# Autodesk Inventor assembly: All Assembly
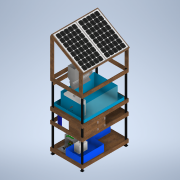
[picture p0: Inventor's stored thumbnail of the model, 180x180]
Saved by Autodesk Inventor 2020 (Build 240168000, 168)
## iProperties
Created: 2020-06-27
Part Number: All Assembly
Document SubType Name: Assembly
Designer: Abbas
Author: Abbas
## Documents named in this file (22)
- C:\Users\LENOVO\Desktop\Graduation Project\Fish Farming Unit\All Assembly\All Assembly.iam
- C:\Users\LENOVO\Desktop\Graduation Project\Fish Farming Unit\tub floor\tub floor 1.ipt
- C:\Users\LENOVO\Desktop\Graduation Project\Fish Farming Unit\tub floor\tub floor 2.ipt
- C:\Users\LENOVO\Desktop\Graduation Project\Fish Farming Unit\metal supporter\metal supporter.ipt
- C:\Users\LENOVO\Desktop\Graduation Project\Fish Farming Unit\Tub\tub_assembled.iam
- C:\Users\LENOVO\Desktop\Graduation Project\Fish Farming Unit\solar panels holder\solar panels holder 2.ipt
- C:\Users\LENOVO\Desktop\Graduation Project\Fish Farming Unit\Solar Panels With Holder\Solar Panels With Holder.iam
- C:\Users\LENOVO\Desktop\Graduation Project\Fish Farming Unit\foodstorage\Assembly1.iam
- C:\Users\LENOVO\Desktop\Graduation Project\Fish Farming Unit\tub floor\tub floor 3.ipt
- C:\Users\LENOVO\Desktop\Graduation Project\Fish Farming Unit\Water Loop Components\Ammonia Filter.iam
- C:\Users\LENOVO\Desktop\Graduation Project\Fish Farming Unit\Middle Floor\Middle Floor.ipt
- C:\Users\LENOVO\Desktop\Graduation Project\Fish Farming Unit\Sensors\NTC Thermistor\NTC thermistor.iam
- C:\Users\LENOVO\Desktop\Graduation Project\Fish Farming Unit\Sensors\ph-sensor-1.snapshot.1\PH_Probe.iam
- C:\Users\LENOVO\Desktop\Graduation Project\Fish Farming Unit\Water Loop Components\ammonia filter bracket.ipt
- C:\Users\LENOVO\Desktop\Graduation Project\Fish Farming Unit\feeding tank bracket\feeding tank bracket.ipt
- C:\Users\LENOVO\Desktop\Graduation Project\Fish Farming Unit\Tub Sensors Holder\Sensors Holder V3.ipt
- C:\Users\LENOVO\Desktop\Graduation Project\Fish Farming Unit\Pump System\Pump System.iam
- C:\Users\LENOVO\Desktop\Graduation Project\Fish Farming Unit\Water Loop Components\Storage_tank.ipt
- C:\Users\LENOVO\Desktop\Graduation Project\Fish Farming Unit\Hinge\Peice 1.ipt
- C:\Users\LENOVO\Desktop\Graduation Project\Fish Farming Unit\Electric Box Covers\Battery Cover.iam
- C:\Users\LENOVO\Desktop\Graduation Project\Fish Farming Unit\Electric Box Covers\Control Cover.iam
- C:\Users\LENOVO\Desktop\Graduation Project\Fish Farming Unit\Ammonia Filter Tub\Ammonia Filter Tub.iam
## Components (28 placed, 22 different names)
1. Solar Panels With Holder:1 [sub-assembly] — Mate:5, Mate:6
2. solar panels holder 2:1 — Insert:11, Insert:12, Mate:5, Mate:6
3. metal supporter:1 — Insert:1, Insert:2, Insert:14, Insert:15
4. metal supporter:2 — Insert:3, Insert:4, Insert:9, Insert:10, Insert:11, Insert:12, Mate:40
5. metal supporter:3 — Insert:7, Insert:8, Insert:21, Insert:22
6. metal supporter:4 — Insert:5, Insert:6
7. tub floor 1:2 — Mate:1, Mate:2, Insert:1, Insert:2, Insert:3, Insert:4, Insert:5, Insert:6, Insert:7, Insert:8, Mate:28
8. tub floor 2:1 — Mate:1, Mate:2, Mate:3, Mate:4, Mate:29
9. tub_assembled:1 [sub-assembly] — Mate:3, Mate:4, Insert:17, Insert:18, Mate:23, Mate:25
10. Assembly1:1 [sub-assembly] — Mate:22, Insert:23
11. feeding tank bracket:1 — Insert:21, Insert:22, Mate:22, Insert:23
12. Middle Bracket — Insert:14, Insert:15, Mate:33, Insert:24, Mate:34, Insert:26, Mate:35, Insert:27, Insert:28, Insert:29
13. Base Bracket — Insert:9, Insert:10, Mate:8, Mate:9
14. Base Floor — Mate:8, Mate:9, Mate:30, Mate:31, Mate:32, Mate:38, Mate:39
15. NTC thermistor:1 [sub-assembly] — Insert:17
16. PH_Probe:1 [sub-assembly] — Insert:18
17. ammonia filter bracket:1 — Insert:19, Mate:28, Mate:29
18. Ammonia Filter:1 [sub-assembly] — Insert:19
19. Sensors Holder V3:1 — Mate:23, Mate:25
20. Pump System:1 [sub-assembly] — Mate:30
21. Storage_tank:1 — Mate:31, Mate:32
22. Peice 1:1 — Mate:33, Insert:24, Insert:25
23. Battery Cover:1 [sub-assembly] — Insert:25
24. Peice 1:2 — Mate:34, Insert:26
25. Peice 1:3 — Mate:35, Insert:27, Insert:30
26. Peice 1:4 — Insert:28, Insert:29
27. Control Cover:1 [sub-assembly] — Insert:30
28. Ammonia Filter Tub:1 [sub-assembly] — Mate:38, Mate:39, Mate:40
## Relationships (49: Insert 27, Mate 22)
- Mate:1: tub floor 1:2 ↔ tub floor 2:1
- Mate:2: tub floor 1:2 ↔ tub floor 2:1
- Insert:1: metal supporter:1 ↔ tub floor 1:2
- Insert:2: metal supporter:1 ↔ tub floor 1:2
- Insert:3: metal supporter:2 ↔ tub floor 1:2
- Insert:4: metal supporter:2 ↔ tub floor 1:2
- Insert:5: metal supporter:4 ↔ tub floor 1:2
- Insert:6: metal supporter:4 ↔ tub floor 1:2
- Insert:7: metal supporter:3 ↔ tub floor 1:2
- Insert:8: metal supporter:3 ↔ tub floor 1:2
- Insert:9: metal supporter:2 ↔ Base Bracket
- Insert:10: metal supporter:2 ↔ Base Bracket
- Mate:3: tub floor 2:1 ↔ tub_assembled:1
- Mate:4: tub floor 2:1 ↔ tub_assembled:1
- Insert:11: solar panels holder 2:1 ↔ metal supporter:2
- Insert:12: solar panels holder 2:1 ↔ metal supporter:2
- Mate:5: Solar Panels With Holder:1 ↔ solar panels holder 2:1
- Mate:6: Solar Panels With Holder:1 ↔ solar panels holder 2:1
- Mate:8: Base Bracket ↔ Base Floor
- Mate:9: Base Bracket ↔ Base Floor
- Insert:14: metal supporter:1 ↔ Middle Bracket
- Insert:15: metal supporter:1 ↔ Middle Bracket
- Insert:17 (-15 mm): tub_assembled:1 ↔ NTC thermistor:1
- Insert:18 (-100 mm): tub_assembled:1 ↔ PH_Probe:1
- Insert:19 (12 mm): ammonia filter bracket:1 ↔ Ammonia Filter:1
- Insert:21: metal supporter:3 ↔ feeding tank bracket:1
- Insert:22: metal supporter:3 ↔ feeding tank bracket:1
- Mate:22: Assembly1:1 ↔ feeding tank bracket:1
- Insert:23: Assembly1:1 ↔ feeding tank bracket:1
- Mate:23: tub_assembled:1 ↔ Sensors Holder V3:1
- Mate:25: tub_assembled:1 ↔ Sensors Holder V3:1
- Mate:28: tub floor 1:2 ↔ ammonia filter bracket:1
- Mate:29: tub floor 2:1 ↔ ammonia filter bracket:1
- Mate:30: Base Floor ↔ Pump System:1
- Mate:31: Base Floor ↔ Storage_tank:1
- Mate:32: Base Floor ↔ Storage_tank:1
- Mate:33: Middle Bracket ↔ Peice 1:1
- Insert:24: Middle Bracket ↔ Peice 1:1
- Insert:25: Peice 1:1 ↔ Battery Cover:1
- Mate:34: Middle Bracket ↔ Peice 1:2
- Insert:26: Middle Bracket ↔ Peice 1:2
- Mate:35: Middle Bracket ↔ Peice 1:3
- Insert:27: Middle Bracket ↔ Peice 1:3
- Insert:28: Middle Bracket ↔ Peice 1:4
- Insert:29: Middle Bracket ↔ Peice 1:4
- Insert:30: Peice 1:3 ↔ Control Cover:1
- Mate:38: Base Floor ↔ Ammonia Filter Tub:1
- Mate:39: Base Floor ↔ Ammonia Filter Tub:1
- Mate:40: metal supporter:2 ↔ Ammonia Filter Tub:1
